# Autodesk Inventor assembly: Ensamblaje1
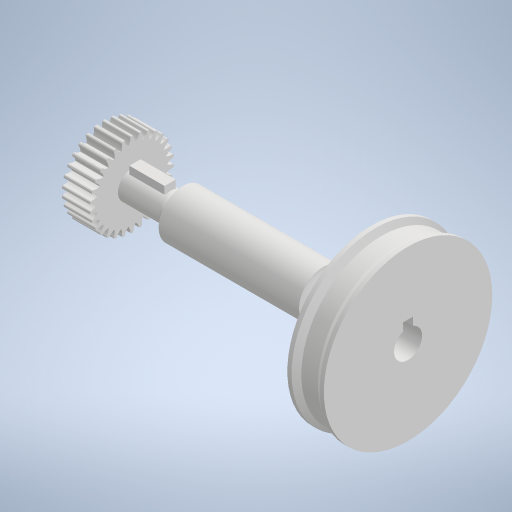
[picture p0: Inventor's stored thumbnail of the model, 512x512]
Saved by Autodesk Inventor 2024 (Build 280153000, 153)
## iProperties
Created: 2024-03-31
Part Number: Ensamblaje1
Document SubType Name: Assembly
Designer: ADRIANA MORALES
Author: ADRIANA MORALES
## Documents named in this file (5)
- C:\Users\ADRIANA MORALES\Documents\DINAMICA PIEZAS\Ensamblaje1.iam
- C:\Users\ADRIANA MORALES\Documents\DINAMICA PIEZAS\EJE_CUÑEROS.ipt
- C:\Users\ADRIANA MORALES\Documents\DINAMICA PIEZAS\ENGRANE.ipt
- C:\Users\ADRIANA MORALES\Documents\DINAMICA PIEZAS\POLEA.ipt
- C:\Users\ADRIANA MORALES\Documents\DINAMICA PIEZAS\CUÑA (1).ipt
## Components (5 placed, 4 different names)
1. EJE_CUÑEROS:1 — Coincidencia:1, Rígido:1, Rígido:2, De rotación:1
2. ENGRANE:1 — De rotación:1
3. POLEA:1 — Coincidencia:1
4. CUÑA (1):1 — Rígido:1
5. CUÑA (1):5 — Rígido:2
## Relationships (4: WeldJoint 2, Mate 1, RevoluteJoint 1)
- Coincidencia:1 [Mate]: EJE_CUÑEROS:1 ↔ POLEA:1
- Rígido:1 [WeldJoint]: EJE_CUÑEROS:1 ↔ CUÑA (1):1
- Rígido:2 [WeldJoint]: EJE_CUÑEROS:1 ↔ CUÑA (1):5
- De rotación:1 [RevoluteJoint]: EJE_CUÑEROS:1 ↔ ENGRANE:1
